# Autodesk Inventor assembly: structure
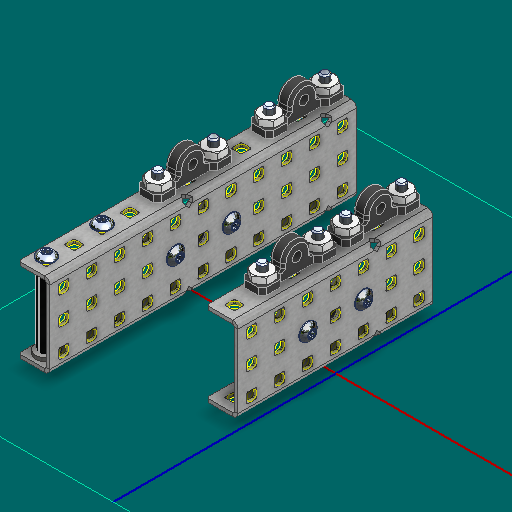
[picture p0: Inventor's stored thumbnail of the model, 512x512]
Saved by Autodesk Inventor 2025 (Build 290162000, 162)
## iProperties
Created: 2024-08-16
Part Number: structure
Document SubType Name: Assembly
Designer: averey
Author: averey
## Documents named in this file (17)
- C:\Users\avere\vex_robotics_high_stakes\hardware\cad\ATLAS\chassis\drive_pod\back_right\structure.iam
- C:\Users\avere\vex_robotics_high_stakes\hardware\cad\VEX-CAD-Inventor\Structure\C Channel\Aluminum 1x3x1\Alu C 1x3x1x7.ipt
- C:\Users\avere\vex_robotics_high_stakes\hardware\cad\_quick_assemblies\bearing_flat_w_hardware.iam
- C:\Users\avere\vex_robotics_high_stakes\hardware\cad\VEX-CAD-Inventor\Structure\C Channel\Aluminum 1x3x1\Alu C 1x3x1x11.ipt
- C:\Users\avere\vex_robotics_high_stakes\hardware\cad\VEX-CAD-Inventor\Motion\Shaft LS\LS Pillow Bearing Block.ipt
- C:\Users\avere\vex_robotics_high_stakes\hardware\cad\VEX-CAD-Inventor\Structure\Hardware\Screw Shoulder Robosource\SScrew Shoulder Smooth .500 x .18.ipt
- C:\Users\avere\vex_robotics_high_stakes\hardware\cad\VEX-CAD-Inventor\Structure\Hardware\Screw Shoulder Robosource.ipt
- C:\Users\avere\vex_robotics_high_stakes\hardware\cad\VEX-CAD-Inventor\Structure\Standoff\Standoff 1.00.ipt
- C:\Users\avere\vex_robotics_high_stakes\hardware\cad\VEX-CAD-Inventor\Structure\Standoff.ipt
- C:\Users\avere\vex_robotics_high_stakes\hardware\cad\VEX-CAD-Inventor\Motion\Spacers\Spacer Nylon .375 OD\NSpacer .375 OD x .125.ipt
- C:\Users\avere\vex_robotics_high_stakes\hardware\cad\VEX-CAD-Inventor\Motion\Spacers\Spacer Nylon .375 OD.ipt
- C:\Users\avere\vex_robotics_high_stakes\hardware\cad\VEX-CAD-Inventor\Structure\Hardware\Screw Shoulder Robosource\SScrew Shoulder Smooth .500 x .04.ipt
- C:\Users\avere\vex_robotics_high_stakes\hardware\cad\VEX-CAD-Inventor\Structure\Standoff\Standoff 1.25.ipt
- C:\Users\avere\vex_robotics_high_stakes\hardware\cad\VEX-CAD-Inventor\Motion\Spacers\Washer Steel\SWasher .375 OD x .062500.ipt
- C:\Users\avere\vex_robotics_high_stakes\hardware\cad\VEX-CAD-Inventor\Motion\Spacers\Washer Steel.ipt
- C:\Users\avere\vex_robotics_high_stakes\hardware\cad\VEX-CAD-Inventor\Structure\Hardware\Nut Nylon\Nut Nylon - White.ipt
- C:\Users\avere\vex_robotics_high_stakes\hardware\cad\VEX-CAD-Inventor\Structure\Hardware\Nut Nylon.ipt
## Components (33 placed, 11 different names)
1. Alu C 1x3x1x7:1 — Mate:1, Insert:1, Mate:2, Insert:2, Mate:3, Insert:9, Mate:10, Insert:10, Mate:11, Insert:20, Insert:21, Insert:22, Insert:23
2. bearing_flat_w_hardware:1 [sub-assembly] — Insert:1, Mate:2
3. Alu C 1x3x1x11:1 — Insert:2, Mate:3, Insert:3, Mate:4, Insert:7, Mate:8, Insert:8, Mate:9, Insert:12, Insert:13, Insert:14, Insert:17, Insert:18, Insert:19, Insert:29, Insert:31, Insert:33, Insert:35
4. bearing_flat_w_hardware:2 [sub-assembly] — Insert:3, Mate:4
5. LS Pillow Bearing Block:1 — Insert:10, Mate:11, Insert:26, Insert:27
6. LS Pillow Bearing Block:2 — Insert:9, Mate:10, Insert:24, Insert:25
7. LS Pillow Bearing Block:3 — Insert:8, Mate:9
8. LS Pillow Bearing Block:4 — Insert:7, Mate:8
9. SScrew Shoulder Smooth .500 x .18:1 — Insert:13
10. Standoff 1.00:1
11. NSpacer .375 OD x .125:1 — Insert:12
12. SScrew Shoulder Smooth .500 x .04:2 — Insert:14
13. Standoff 1.25:1
14. SWasher .375 OD x .062500:1 — Insert:17
15. SWasher .375 OD x .062500:2
16. SScrew Shoulder Smooth .500 x .18:3 — Insert:18
17. SScrew Shoulder Smooth .500 x .18:4 — Insert:19
18. SScrew Shoulder Smooth .500 x .18:5 — Insert:20
19. SScrew Shoulder Smooth .500 x .18:6 — Insert:21
20. SScrew Shoulder Smooth .500 x .18:7 — Insert:23
21. SScrew Shoulder Smooth .500 x .18:8 — Insert:22
22. Nut Nylon - White:1 — Insert:25
23. Nut Nylon - White:2 — Insert:24
24. Nut Nylon - White:3 — Insert:26
25. Nut Nylon - White:4 — Insert:27
26. SScrew Shoulder Smooth .500 x .18:9 — Insert:28, Insert:29
27. Nut Nylon - White:5 — Insert:28
28. SScrew Shoulder Smooth .500 x .18:10 — Insert:31
29. Nut Nylon - White:6
30. SScrew Shoulder Smooth .500 x .18:11 — Insert:33
31. Nut Nylon - White:7
32. SScrew Shoulder Smooth .500 x .18:12 — Insert:35
33. Nut Nylon - White:8
## Relationships (40: Insert 32, Mate 8)
- Mate:1: Alu C 1x3x1x7:1
- Insert:1: Alu C 1x3x1x7:1 ↔ bearing_flat_w_hardware:1
- Mate:2: Alu C 1x3x1x7:1 ↔ bearing_flat_w_hardware:1
- Insert:2 (58.7375 mm): Alu C 1x3x1x7:1 ↔ Alu C 1x3x1x11:1
- Mate:3: Alu C 1x3x1x7:1 ↔ Alu C 1x3x1x11:1
- Insert:3: Alu C 1x3x1x11:1 ↔ bearing_flat_w_hardware:2
- Mate:4: Alu C 1x3x1x11:1 ↔ bearing_flat_w_hardware:2
- Insert:7 (1.5875 mm): Alu C 1x3x1x11:1 ↔ LS Pillow Bearing Block:4
- Mate:8: Alu C 1x3x1x11:1 ↔ LS Pillow Bearing Block:4
- Insert:8 (1.5875 mm): Alu C 1x3x1x11:1 ↔ LS Pillow Bearing Block:3
- Mate:9: Alu C 1x3x1x11:1 ↔ LS Pillow Bearing Block:3
- Insert:9 (1.5875 mm): Alu C 1x3x1x7:1 ↔ LS Pillow Bearing Block:2
- Mate:10: Alu C 1x3x1x7:1 ↔ LS Pillow Bearing Block:2
- Insert:10 (1.5875 mm): Alu C 1x3x1x7:1 ↔ LS Pillow Bearing Block:1
- Mate:11: Alu C 1x3x1x7:1 ↔ LS Pillow Bearing Block:1
- [Insert]: Standoff 1.00:1 ↔ NSpacer .375 OD x .125:1
- Insert:12: Alu C 1x3x1x11:1 ↔ NSpacer .375 OD x .125:1
- Insert:13 (1.5875 mm): Alu C 1x3x1x11:1 ↔ SScrew Shoulder Smooth .500 x .18:1
- Insert:14 (1.5875 mm): Alu C 1x3x1x11:1 ↔ SScrew Shoulder Smooth .500 x .04:2
- [Insert]: Standoff 1.25:1 ↔ SWasher .375 OD x .062500:1
- [Insert]: Standoff 1.25:1 ↔ SWasher .375 OD x .062500:2
- Insert:17: Alu C 1x3x1x11:1 ↔ SWasher .375 OD x .062500:1
- Insert:18 (1.5875 mm): Alu C 1x3x1x11:1 ↔ SScrew Shoulder Smooth .500 x .18:3
- Insert:19 (1.5875 mm): Alu C 1x3x1x11:1 ↔ SScrew Shoulder Smooth .500 x .18:4
- Insert:20: Alu C 1x3x1x7:1 ↔ SScrew Shoulder Smooth .500 x .18:5
- Insert:21: Alu C 1x3x1x7:1 ↔ SScrew Shoulder Smooth .500 x .18:6
- Insert:22: Alu C 1x3x1x7:1 ↔ SScrew Shoulder Smooth .500 x .18:8
- Insert:23: Alu C 1x3x1x7:1 ↔ SScrew Shoulder Smooth .500 x .18:7
- Insert:24: LS Pillow Bearing Block:2 ↔ Nut Nylon - White:2
- Insert:25: LS Pillow Bearing Block:2 ↔ Nut Nylon - White:1
- Insert:26: LS Pillow Bearing Block:1 ↔ Nut Nylon - White:3
- Insert:27: LS Pillow Bearing Block:1 ↔ Nut Nylon - White:4
- Insert:28 (6.35 mm): SScrew Shoulder Smooth .500 x .18:9 ↔ Nut Nylon - White:5
- Insert:29: Alu C 1x3x1x11:1 ↔ SScrew Shoulder Smooth .500 x .18:9
- [Insert] (6.35 mm): SScrew Shoulder Smooth .500 x .18:10 ↔ Nut Nylon - White:6
- Insert:31: Alu C 1x3x1x11:1 ↔ SScrew Shoulder Smooth .500 x .18:10
- [Insert] (6.35 mm): SScrew Shoulder Smooth .500 x .18:11 ↔ Nut Nylon - White:7
- Insert:33: Alu C 1x3x1x11:1 ↔ SScrew Shoulder Smooth .500 x .18:11
- [Insert] (6.35 mm): SScrew Shoulder Smooth .500 x .18:12 ↔ Nut Nylon - White:8
- Insert:35: Alu C 1x3x1x11:1 ↔ SScrew Shoulder Smooth .500 x .18:12
## Named parameters: d40_d33 = 0 mm, d41_d34 = 0 mm, d46_d44 = 6.35 mm, d48_d44 = 6.35 mm, d51_d48_d44 = 6.35 mm
